# Autodesk Inventor assembly: frame assembly
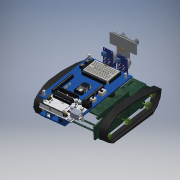
[picture p0: Inventor's stored thumbnail of the model, 180x180]
Saved by Autodesk Inventor 2017 (Build 210142000, 142)
## iProperties
Created: 2019-12-31
Part Number: frame assembly
Document SubType Name: Assembly
Designer: Admin
Author: Admin
## Documents named in this file (15)
- D:\tech design 11\1 New Robot\CAd\frame assembly.iam
- D:\tech design 11\1 New Robot\CAd\side frame.ipt
- D:\tech design 11\1 New Robot\CAd\top bottom frame.ipt
- D:\tech design 11\1 New Robot\CAd\top frame 4x4.ipt
- D:\tech design 11\1 New Robot\CAd\boeshield.ipt
- D:\tech design 11\1 New Robot\CAd\Wheels.ipt
- D:\tech design 11\1 New Robot\CAd\track.ipt
- D:\tech design 11\1 New Robot\CAd\arduinoUnoDetailed.ipt
- D:\tech design 11\1 New Robot\CAd\MQ135_sensor.ipt
- D:\tech design 11\1 New Robot\CAd\Buzzer_Active.ipt
- D:\tech design 11\1 New Robot\CAd\Electronics_Prototyping_Breadboard_35x45x8_17x10holes.ipt
- D:\tech design 11\1 New Robot\CAd\Tower Pro MG90S Micro servo.iam
- D:\tech design 11\1 New Robot\CAd\hc-sr04.ipt
- D:\tech design 11\1 New Robot\CAd\Parallax Servo 900-00005.iam
- D:\tech design 11\1 New Robot\CAd\ultrasonic_sensor_ho.ipt
## Components (30 placed, 14 different names)
1. side frame:1 — Mate:4, Mate:5, Mate:6, Mate:7, Insert:1, Insert:2, Insert:3, Insert:4, Insert:5, Symmetry:1
2. top bottom frame:1 — Mate:7, Mate:8, Mate:9, Mate:10, Mate:13, Mate:14
3. top frame 4x4:1 — Mate:1, Mate:2, Mate:3, Mate:4, Mate:5, Mate:6, Mate:11, Mate:18, Mate:20
4. side frame:2 — Mate:1, Mate:2, Mate:3, Mate:8, Mate:9, Mate:10, Insert:6, Insert:7, Insert:8, Insert:9, Insert:10, Insert:11, Mate:19
5. boeshield:1 — Mate:11, Mate:12
6. Wheels:6 — Insert:4
7. Wheels:7 — Insert:7
8. Wheels:8 — Insert:6
9. Wheels:9 — Insert:3
10. Wheels:10 — Insert:1
11. Wheels:11 — Insert:2, Symmetry:1, Mate:21
12. Wheels:12 — Insert:5
13. Wheels:13 — Insert:10
14. Wheels:14 — Insert:9
15. Wheels:15 — Insert:8
16. Wheels:16 — Insert:11
17. Wheels:17
18. track:1
19. track:3
20. arduinoUnoDetailed:1 — Mate:12
21. MQ135_sensor:1 — Mate:15
22. Buzzer_Active:1
23. MQ135_sensor:2 — Mate:16
24. MQ135_sensor:3
25. Electronics_Prototyping_Breadboard_35x45x8_17x10holes:1 — Mate:13, Mate:14, Mate:15, Mate:16, Mate:17
26. Tower Pro MG90S Micro servo:1 [sub-assembly] — Mate:17, Insert:12
27. hc-sr04:1 — Mate:22
28. Parallax Servo 900-00005:1 [sub-assembly] — Mate:18, Mate:19
29. Parallax Servo 900-00005:2 [sub-assembly] — Mate:20, Mate:21
30. ultrasonic_sensor_ho:1 — Insert:12, Mate:22
## Relationships (35: Mate 22, Insert 12, Symmetry 1)
- Mate:1: top frame 4x4:1 ↔ side frame:2
- Mate:2: top frame 4x4:1 ↔ side frame:2
- Mate:3: top frame 4x4:1 ↔ side frame:2
- Mate:4: side frame:1 ↔ top frame 4x4:1
- Mate:5: side frame:1 ↔ top frame 4x4:1
- Mate:6: side frame:1 ↔ top frame 4x4:1
- Mate:7: side frame:1 ↔ top bottom frame:1
- Mate:8: top bottom frame:1 ↔ side frame:2
- Mate:9: top bottom frame:1 ↔ side frame:2
- Mate:10: top bottom frame:1 ↔ side frame:2
- Mate:11: top frame 4x4:1 ↔ boeshield:1
- Insert:1: side frame:1 ↔ Wheels:10
- Insert:2: side frame:1 ↔ Wheels:11
- Insert:3: side frame:1 ↔ Wheels:9
- Insert:4: side frame:1 ↔ Wheels:6
- Insert:5: side frame:1 ↔ Wheels:12
- Insert:6: side frame:2 ↔ Wheels:8
- Insert:7: side frame:2 ↔ Wheels:7
- Insert:8: side frame:2 ↔ Wheels:15
- Insert:9: side frame:2 ↔ Wheels:14
- Insert:10: side frame:2 ↔ Wheels:13
- Insert:11: side frame:2 ↔ Wheels:16
- Symmetry:1: side frame:1 ↔ Wheels:11
- Mate:12: boeshield:1 ↔ arduinoUnoDetailed:1
- Mate:13: top bottom frame:1 ↔ Electronics_Prototyping_Breadboard_35x45x8_17x10holes:1
- Mate:14: top bottom frame:1 ↔ Electronics_Prototyping_Breadboard_35x45x8_17x10holes:1
- Mate:15: MQ135_sensor:1 ↔ Electronics_Prototyping_Breadboard_35x45x8_17x10holes:1
- Mate:16: MQ135_sensor:2 ↔ Electronics_Prototyping_Breadboard_35x45x8_17x10holes:1
- Mate:17: Electronics_Prototyping_Breadboard_35x45x8_17x10holes:1 ↔ Tower Pro MG90S Micro servo:1
- Mate:18: top frame 4x4:1 ↔ Parallax Servo 900-00005:1
- Mate:19: side frame:2 ↔ Parallax Servo 900-00005:1
- Mate:20: top frame 4x4:1 ↔ Parallax Servo 900-00005:2
- Mate:21: Wheels:11 ↔ Parallax Servo 900-00005:2
- Insert:12: Tower Pro MG90S Micro servo:1 ↔ ultrasonic_sensor_ho:1
- Mate:22: hc-sr04:1 ↔ ultrasonic_sensor_ho:1
